# Autodesk Inventor assembly: bisonV2
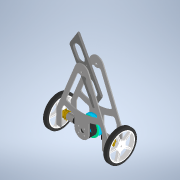
[picture p0: Inventor's stored thumbnail of the model, 180x180]
Saved by Autodesk Inventor 2021 (Build 250183000, 183)
## iProperties
Created: 2022-10-22
Part Number: bisonV2
Document SubType Name: Assembly
Designer: ermoz
Author: ermoz
## Documents named in this file (8)
- D:\Moje Wyczyny\My_Poor_Projects\combat-bison\mechanics\bisonV2.iam
- D:\Moje Wyczyny\My_Poor_Projects\combat-bison\mechanics\redox_bl_400_1400.ipt
- D:\Moje Wyczyny\My_Poor_Projects\combat-bison\mechanics\wheel.ipt
- D:\Moje Wyczyny\My_Poor_Projects\combat-bison\mechanics\Pololu_MicroMotor.ipt
- D:\Moje Wyczyny\My_Poor_Projects\combat-bison\mechanics\rotorV2.ipt
- D:\Moje Wyczyny\My_Poor_Projects\combat-bison\mechanics\motor_gear.ipt
- D:\Moje Wyczyny\My_Poor_Projects\combat-bison\mechanics\frame_rotor.ipt
- D:\Moje Wyczyny\My_Poor_Projects\combat-bison\mechanics\motor_gear_end.ipt
## Components (10 placed, 7 different names)
1. redox_bl_400_1400:1 — Mate:1, Mate:2, Mate:3, Mate:8, Mate:9, Mate:10, Mate:12, Mate:15
2. wheel:1 — Mate:4, Mate:6, Mate:14
3. wheel:2 — Mate:5, Mate:7, Mate:14
4. Pololu_MicroMotor:1 — Mate:5, Mate:7
5. Pololu_MicroMotor:2 — Mate:4, Mate:6
6. rotorV2:1 — Mate:11, Mate:13
7. motor_gear:1 — Mate:1, Mate:2, Mate:3, Mate:16
8. frame_rotor:1 — Mate:8, Mate:9, Mate:10, Mate:11
9. frame_rotor:2 — Mate:12, Mate:13
10. motor_gear_end:1 — Mate:15, Mate:16
## Relationships (16: Mate 16)
- Mate:1: redox_bl_400_1400:1 ↔ motor_gear:1
- Mate:2: redox_bl_400_1400:1 ↔ motor_gear:1
- Mate:3: redox_bl_400_1400:1 ↔ motor_gear:1
- Mate:4: wheel:1 ↔ Pololu_MicroMotor:2
- Mate:5: wheel:2 ↔ Pololu_MicroMotor:1
- Mate:6: wheel:1 ↔ Pololu_MicroMotor:2
- Mate:7: wheel:2 ↔ Pololu_MicroMotor:1
- Mate:8: redox_bl_400_1400:1 ↔ frame_rotor:1
- Mate:9: redox_bl_400_1400:1 ↔ frame_rotor:1
- Mate:10: redox_bl_400_1400:1 ↔ frame_rotor:1
- Mate:11: rotorV2:1 ↔ frame_rotor:1
- Mate:12: redox_bl_400_1400:1 ↔ frame_rotor:2
- Mate:13: rotorV2:1 ↔ frame_rotor:2
- Mate:14: wheel:1 ↔ wheel:2
- Mate:15: redox_bl_400_1400:1 ↔ motor_gear_end:1
- Mate:16: motor_gear:1 ↔ motor_gear_end:1
